# Autodesk Inventor assembly: Giant-Snes-Gamepad
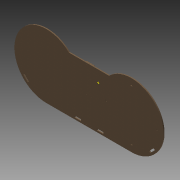
[picture p0: Inventor's stored thumbnail of the model, 180x180]
Saved by Autodesk Inventor 2014 SP1 (Build 180222100, 222)
## iProperties
Created: 2014-01-12
Part Number: Giant-Snes-Gamepad
Document SubType Name: Assembly
Designer: tuleu
Author: tuleu
## Documents named in this file (4)
- C:\Users\tuleu\Documents\giant-snes-gamepad\cad\Giant_Snes_Gamepad.iam
- C:\Users\tuleu\Documents\giant-snes-gamepad\cad\Link.ipt
- C:\Users\tuleu\Documents\giant-snes-gamepad\cad\Gamepad_Left.iam
- C:\Users\tuleu\Documents\giant-snes-gamepad\cad\Gamepad_Right.iam
## Components (5 placed, 3 different names)
1. Link:1
2. Link:2 — Mate:14
3. Link:3
4. Gamepad_Left:1 [sub-assembly]
5. Gamepad_Right:1 [sub-assembly]
## Relationships (21: Mate 15, Flush 4, Angle 2)
- [Mate]: Gamepad_Left:1 ↔ Gamepad_Right:1
- [Mate]: Gamepad_Left:1 ↔ Gamepad_Right:1
- [Flush]: Gamepad_Left:1 ↔ Gamepad_Right:1
- [Mate]: Gamepad_Left:1 ↔ Gamepad_Right:1
- [Mate]: Link:1 ↔ Gamepad_Right:1
- [Mate]: Link:2 ↔ Gamepad_Left:1
- [Mate]: Link:3 ↔ Gamepad_Left:1
- [Flush]: Link:1 ↔ Gamepad_Right:1
- [Flush]: Link:3 ↔ Gamepad_Left:1
- [Mate]: Link:2 ↔ Gamepad_Right:1
- [Mate]: Link:3 ↔ Gamepad_Right:1
- [Mate]: Link:1 ↔ Gamepad_Right:1
- [Mate]: Gamepad_Right:1
- Mate:14: Link:2
- [Mate] (-205 mm): Gamepad_Left:1
- [Mate]: Gamepad_Left:1
- [Angle] (0 deg): Gamepad_Left:1
- [Mate]: Gamepad_Left:1
- [Mate]: Gamepad_Right:1
- [Angle] (0 deg): Gamepad_Left:1
- [Flush]: Gamepad_Right:1
